# Autodesk Inventor assembly: ForeArmAssembly
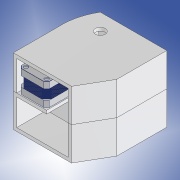
[picture p0: Inventor's stored thumbnail of the model, 180x180]
Saved by Autodesk Inventor 2017 (Build 210142000, 142)
## iProperties
Created: 2017-06-14
Part Number: ForeArmAssembly
Document SubType Name: Assembly
Designer: zallen
Author: zallen
## Documents named in this file (4)
- C:\Users\zallen\Documents\GitHub\cr-laundry-robot\src\Body\Arm Assembly\Fore Arm Assembly\ForeArmAssembly.iam
- C:\Users\zallen\Documents\GitHub\cr-laundry-robot\src\Body\Arm Assembly\Fore Arm Assembly\FA001.ipt
- C:\Users\zallen\Documents\GitHub\cr-laundry-robot\src\Body\Arm Assembly\Fore Arm Assembly\FA002.ipt
- C:\Users\zallen\Documents\GitHub\cr-laundry-robot\lib\Stepper Motor - NEMA 17\NEMA17.ipt
## Components (3 placed, 3 different names)
1. FA001:1 — Mate:1, Mate:3, Mate:4, Mate:5, Mate:6
2. FA002:1 — Mate:1, Mate:4
3. NEMA17:1 — Mate:3, Mate:5, Mate:6
## Relationships (5: Mate 5)
- Mate:1: FA001:1 ↔ FA002:1
- Mate:3: FA001:1 ↔ NEMA17:1
- Mate:4: FA001:1 ↔ FA002:1
- Mate:5: FA001:1 ↔ NEMA17:1
- Mate:6: FA001:1 ↔ NEMA17:1
